# Autodesk Inventor assembly: MuRail
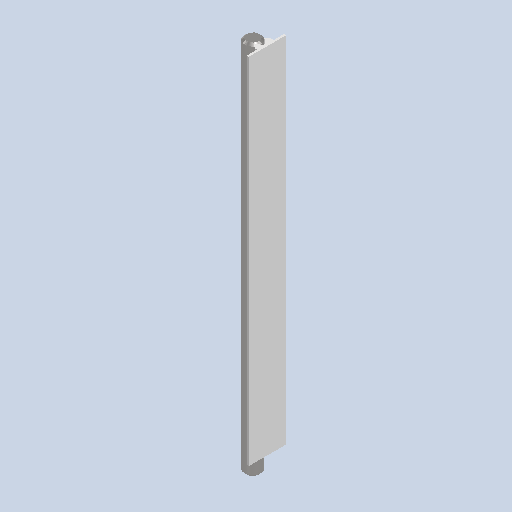
[picture p0: Inventor's stored thumbnail of the model, 512x512]
Saved by Autodesk Inventor 2024 (Build 280153000, 153)
## iProperties
Created: 2023-08-21
Part Number: MuRail
Document SubType Name: Assembly
Designer: KirikDK
Author: KirikDK
## Documents named in this file (3)
- C:\WorkProject\CNC_Lathe\MiniTocatka\MuRail.iam
- C:\WorkProject\CNC_Lathe\MiniTocatka\RailDerzavka.ipt
- C:\WorkProject\CNC_Lathe\MiniTocatka\Val340.ipt
## Components (2 placed, 2 different names)
1. RailDerzavka:1 — Flush:1
2. Val340:1 — Flush:1
## Relationships (1: Flush 1)
- Flush:1: RailDerzavka:1 ↔ Val340:1
